# Autodesk Inventor assembly: Mark 3.5
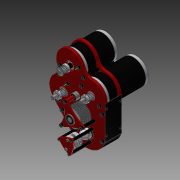
[picture p0: Inventor's stored thumbnail of the model, 180x180]
Saved by Autodesk Inventor 2013 (Build 170138000, 138)
## iProperties
Created: 2013-06-27
Part Number: Mark 3.5
Document SubType Name: Assembly
Designer: mvarma
Author: mvarma
## Documents named in this file (58)
- C:\Users\mvarma\Desktop\GRT 2013-2014 Gearbox\Mark 3\Mark 3.5.iam
- C:\Users\mvarma\Desktop\GRT 2013-2014 Gearbox\Mark 3\Plates\Mounting Plate.ipt
- C:\Users\mvarma\Desktop\GRT 2013-2014 Gearbox\Mark 3\Plates\Pnuematic Plate.ipt
- C:\Users\mvarma\Desktop\GRT 2013-2014 Gearbox\Mark 3\Plates\Main Connecting Standoff.ipt
- C:\Users\mvarma\Desktop\GRT 2013-2014 Gearbox\Mark 3\Pem Nuts\10-32 Clinch Style Pem Nut .091 Minimum Panel Thickness.ipt
- C:\Users\mvarma\Desktop\GRT 2013-2014 Gearbox\Mark 3\Bearings\FR8-2RS.ipt
- C:\Users\mvarma\Desktop\GRT 2013-2014 Gearbox\Mark 3\Bearings\FR6-2RS.ipt
- C:\Users\mvarma\Desktop\GRT 2013-2014 Gearbox\Mark 3\Encoder\Encoder Mount.ipt
- C:\Users\mvarma\Desktop\GRT 2013-2014 Gearbox\Mark 3\Encoder\S4-120-250-N-S-B.ipt
- C:\Users\mvarma\Desktop\GRT 2013-2014 Gearbox\Mark 3\Shafts\Flexible Shaft Coupler 6208K411.ipt
- C:\Users\mvarma\Desktop\GRT 2013-2014 Gearbox\Mark 3\Shafts\Cluster Shaft.ipt
- C:\Users\mvarma\Desktop\GRT 2013-2014 Gearbox\Mark 3\Spacers\Cluster Shaft Spacer.ipt
- C:\Users\mvarma\Desktop\GRT 2013-2014 Gearbox\Mark 3\Bolts\Socket Head Cap Screw 6-32 Thread 1.500 Length.ipt
- C:\Users\mvarma\Desktop\GRT 2013-2014 Gearbox\Mark 3\Gears\15T 20DP - .375 Hex Bore.ipt
- C:\Users\mvarma\Desktop\GRT 2013-2014 Gearbox\Mark 3\Gears\28T 20DP - .375 Hex Bore.ipt
- C:\Users\mvarma\Desktop\GRT 2013-2014 Gearbox\Mark 3\Bearings\FR6-2ZZ - Hex.ipt
- C:\Users\mvarma\Desktop\GRT 2013-2014 Gearbox\Mark 3\Shafts\Output Shaft.ipt
- C:\Users\mvarma\Desktop\GRT 2013-2014 Gearbox\Mark 3\Spacers\Shim 10 thou .500 Bore.ipt
- C:\Users\mvarma\Desktop\GRT 2013-2014 Gearbox\Mark 3\Bearings\R10-Open.ipt
- C:\Users\mvarma\Desktop\GRT 2013-2014 Gearbox\Mark 3\Gears\35T 20DP - .188 Ball Shifting Bore.ipt
- C:\Users\mvarma\Desktop\GRT 2013-2014 Gearbox\Mark 3\Gears\48T 20DP - .188 Ball Shifting Bore.ipt
- C:\Users\mvarma\Desktop\GRT 2013-2014 Gearbox\Mark 3\Bearings\Thrust Bearing Washer - .6250 Bore.ipt
- C:\Users\mvarma\Desktop\GRT 2013-2014 Gearbox\Mark 3\Spacers\Shim 10 thou .625 Bore.ipt
- C:\Users\mvarma\Desktop\GRT 2013-2014 Gearbox\Mark 3\Shafts\Ball Shifting Shaft.ipt
- C:\Users\mvarma\Desktop\GRT 2013-2014 Gearbox\Mark 3\Shafts\Output Shaft Insert.ipt
- C:\Users\mvarma\Desktop\GRT 2013-2014 Gearbox\Mark 3\Spacers\Shim 10 thou .375 Bore.ipt
- C:\Users\mvarma\Desktop\GRT 2013-2014 Gearbox\Mark 3\Pulleys\48T 3mm GT2 - .375 Hex Broach - Hubless.ipt
- C:\Users\mvarma\Desktop\GRT 2013-2014 Gearbox\Mark 3\Plates\Supporting Plate Standoff.ipt
- C:\Users\mvarma\Desktop\GRT 2013-2014 Gearbox\Mark 3\Bolts\Socket Head Cap Screw 10-32 Thread 3.000 Length.ipt
- C:\Users\mvarma\Desktop\GRT 2013-2014 Gearbox\Mark 3\Shafts\Tensioning Shaft.ipt
- C:\Users\mvarma\Desktop\GRT 2013-2014 Gearbox\Mark 3\Spacers\Belt Shaft Spacer 1.ipt
- C:\Users\mvarma\Desktop\GRT 2013-2014 Gearbox\Mark 3\Spacers\Belt Shaft Spacer 2.ipt
- C:\Users\mvarma\Desktop\GRT 2013-2014 Gearbox\Mark 3\Bearings\R4-2RS.ipt
- C:\Users\mvarma\Desktop\GRT 2013-2014 Gearbox\Mark 3\Bearings\R3-2RS.ipt
- C:\Users\mvarma\Desktop\GRT 2013-2014 Gearbox\Mark 3\Plates\Cim Plate.ipt
- C:\Users\mvarma\Desktop\GRT 2013-2014 Gearbox\Mark 3\Bolts\Socket Head Cap Screw 10-32 Thread 1.750 Length.ipt
- C:\Users\mvarma\Desktop\GRT 2013-2014 Gearbox\Mark 3\Motors\Mini CIM Can.ipt
- C:\Users\mvarma\Desktop\GRT 2013-2014 Gearbox\Mark 3\Motors\CIM Can.ipt
- C:\Users\mvarma\Desktop\GRT 2013-2014 Gearbox\Mark 3\Motors\Rotor.ipt
- C:\Users\mvarma\Desktop\GRT 2013-2014 Gearbox\Mark 3\Bolts\Socket Head Cap Screw 10-32 Thread .750 Length.ipt
- C:\Users\mvarma\Desktop\GRT 2013-2014 Gearbox\Mark 3\Pneumatic\FO_020_318_4F_2_03.iam
- C:\Users\mvarma\Desktop\GRT 2013-2014 Gearbox\Mark 3\Pneumatic\Mouning Standoff.ipt
- C:\Users\mvarma\Desktop\GRT 2013-2014 Gearbox\Mark 3\Pneumatic\Mounting Plate.ipt
- C:\Users\mvarma\Desktop\GRT 2013-2014 Gearbox\Mark 3\Pneumatic\Pneumatic Connector -Actuator Side.ipt
- C:\Users\mvarma\Desktop\GRT 2013-2014 Gearbox\Mark 3\Pneumatic\Pneumatic Connector -Shaft Side Cover.ipt
- C:\Users\mvarma\Desktop\GRT 2013-2014 Gearbox\Mark 3\Pem Nuts\4-40 Clinch Style Pem Nut .091 Minimum Panel Thickness.ipt
- C:\Users\mvarma\Desktop\GRT 2013-2014 Gearbox\Mark 3\Bolts\Socket Head Cap Screw 4-40 Thread 1.000 Length.ipt
- C:\Users\mvarma\Desktop\GRT 2013-2014 Gearbox\Mark 3\.0625 Spring Pin .2500 Long.ipt
- C:\Users\mvarma\Desktop\GRT 2013-2014 Gearbox\Mark 3\Bolts\Button Head Cap Screw 4-40 Thread .125 Length.ipt
- C:\Users\mvarma\Desktop\GRT 2013-2014 Gearbox\Mark 3\Bolts\Socket Head Cap Screw 8-32 Thread .375 Length.ipt
- C:\Users\mvarma\Desktop\GRT 2013-2014 Gearbox\Mark 3\Bolts\Socket Head Cap Screw 6-32 Thread 2.250 Length.ipt
- C:\Users\mvarma\Desktop\GRT 2013-2014 Gearbox\Mark 3\Pulleys\16T 3mm GT2 - 8mm Key Broach.ipt
- C:\Users\mvarma\Desktop\GRT 2013-2014 Gearbox\Mark 3\Spacers\Cim Spacer.ipt
- C:\Users\mvarma\Desktop\GRT 2013-2014 Gearbox\Mark 3\Spacers\MiniCim Spacer.ipt
- C:\Users\mvarma\Desktop\GRT 2013-2014 Gearbox\Mark 3\Pem Nuts\.25-20 Clinch Style Pem Nut .125 Minimum Panel Thickness.ipt
- C:\Users\mvarma\Desktop\GRT 2013-2014 Gearbox\Mark 3\Frame Segment.ipt
- C:\Users\mvarma\Desktop\GRT 2013-2014 Gearbox\Mark 3\Plates\Sheild.ipt
- C:\Users\mvarma\Desktop\GRT 2013-2014 Gearbox\Mark 3\Plates\Sheild - Upper.ipt
## Components (116 placed, 56 different names)
1. 10-32 Clinch Style Pem Nut .091 Minimum Panel Thickness:1 — Mate:24, Mate:31
2. 10-32 Clinch Style Pem Nut .091 Minimum Panel Thickness:2 — Mate:27, Mate:28
3. 10-32 Clinch Style Pem Nut .091 Minimum Panel Thickness:3 — Mate:26, Mate:30
4. 10-32 Clinch Style Pem Nut .091 Minimum Panel Thickness:4 — Mate:33, Mate:238
5. 10-32 Clinch Style Pem Nut .091 Minimum Panel Thickness:5 — Mate:20, Mate:36
6. 10-32 Clinch Style Pem Nut .091 Minimum Panel Thickness:6 — Mate:21, Mate:34
7. 10-32 Clinch Style Pem Nut .091 Minimum Panel Thickness:7 — Mate:23, Mate:29
8. 10-32 Clinch Style Pem Nut .091 Minimum Panel Thickness:8 — Mate:35, Mate:239
9. 10-32 Clinch Style Pem Nut .091 Minimum Panel Thickness:9 — Mate:25, Mate:32
10. FR8-2RS:1 — Mate:37, Mate:40, Mate:65, Mate:67
11. FR6-2RS:1 — Mate:38, Mate:39, Mate:51
12. Encoder Mount:1 — Mate:41, Mate:42, Mate:43, Mate:44, Mate:45, Mate:52, Mate:53, Mate:54, Mate:55
13. S4-120-250-N-S-B:1 — Mate:44, Mate:45, Mate:46, Mate:47, Mate:48
14. Flexible Shaft Coupler 6208K411:1 — Mate:46, Mate:47, Mate:49
15. Cluster Shaft:1 — Mate:48, Mate:49, Mate:50, Mate:56, Mate:57, Mate:58, Mate:59, Mate:62, Mate:63, Mate:88, Mate:90, Mate:91, Mate:92, Mate:93, Mate:94, Mate:95, Mate:98
16. Cluster Shaft Spacer:1 — Mate:50, Mate:51, Mate:60
17. Socket Head Cap Screw 6-32 Thread 1.500 Length:1 — Mate:52, Mate:55
18. Socket Head Cap Screw 6-32 Thread 1.500 Length:2 — Mate:53, Mate:54
19. 15T 20DP - .375 Hex Bore:1 — Mate:56, Mate:58, Mate:61, Mate:64
20. 28T 20DP - .375 Hex Bore:1 — Mate:57, Mate:59, Mate:60, Mate:61
21. FR6-2ZZ - Hex:1 — Mate:62, Mate:63, Mate:64, Mate:89
22. Output Shaft:1 — Mate:65, Mate:66, Mate:68, Mate:69, Mate:71, Mate:72, Mate:74, Mate:76, Mate:79, Mate:81, Mate:83, Mate:84, Mate:86, Mate:87, Mate:235
23. Shim 10 thou .500 Bore:1 — Mate:66, Mate:67, Mate:68, Mate:70
24. R10-Open:1 — Mate:69, Mate:70, Mate:73
25. R10-Open:2 — Mate:76, Mate:77, Mate:78
26. 35T 20DP - .188 Ball Shifting Bore:1 — Mate:71, Mate:73, Mate:75
27. 48T 20DP - .188 Ball Shifting Bore:1 — Mate:72, Mate:78, Mate:80
28. Thrust Bearing Washer - .6250 Bore:1 — Mate:79, Mate:80, Mate:82
29. Thrust Bearing Washer - .6250 Bore:2 — Mate:74, Mate:75, Mate:77
30. Shim 10 thou .625 Bore:1 — Mate:81, Mate:82
31. Ball Shifting Shaft:1 — Mate:85, Flush:1, Mate:123, Mate:124, Mate:196, Mate:198, Mate:199
32. Output Shaft Insert:1 — Mate:83, Mate:84, Mate:85, Flush:1
33. FR8-2RS:2 — Mate:86, Mate:87
34. Shim 10 thou .500 Bore:2 — Mate:88, Mate:89, Mate:96
35. Shim 10 thou .375 Bore:1 — Mate:90, Mate:91, Mate:99
36. 48T 3mm GT2 - .375 Hex Broach - Hubless:1 — Mate:93, Mate:95, Mate:97, Flush:2
37. 48T 3mm GT2 - .375 Hex Broach - Hubless:2 — Mate:92, Mate:94, Mate:96, Mate:97, Mate:223, Mate:224
38. FR6-2RS:2 — Mate:98, Mate:99, Mate:100, Mate:101
39. Supporting Plate Standoff:1 — Mate:103, Mate:106
40. Supporting Plate Standoff:2 — Mate:104, Mate:105
41. Socket Head Cap Screw 10-32 Thread 3.000 Length:1 — Mate:108, Mate:109
42. Socket Head Cap Screw 10-32 Thread 3.000 Length:2 — Mate:111, Mate:112, Mate:113
43. Socket Head Cap Screw 10-32 Thread 3.000 Length:3 — Mate:107, Mate:110
44. Tensioning Shaft:1 — Mate:113, Mate:114, Mate:115, Mate:116, Mate:117, Mate:118
45. Belt Shaft Spacer 1:1 — Mate:115, Mate:120
46. Belt Shaft Spacer 2:1 — Mate:116, Mate:121, Mate:122
47. R4-2RS:1 — Mate:118, Mate:119, Mate:120
48. R4-2RS:2 — Mate:117, Mate:119, Mate:121
49. R3-2RS:1 — Mate:123, Mate:124, Mate:200
50. Cim Plate:1 — Mate:127, Mate:128, Mate:129, Mate:130, Mate:131, Mate:132, Mate:133, Mate:134, Mate:135, Mate:136, Mate:137, Mate:138, Mate:139, Mate:140, Mate:141, Mate:142, Mate:143, Mate:144, Mate:145, Mate:146, Mate:147, Mate:148, Mate:149, Mate:150, Mate:151, Mate:152, Mate:153, Mate:154, Mate:155, Mate:162, Mate:163, Mate:164, Mate:165, Mate:166, Mate:167, Mate:168, Mate:169, Mate:170, Mate:171, Mate:172, Mate:173, Mate:174, Mate:175, Mate:176, Mate:177, Mate:178, Mate:179, Mate:242, Mate:243, Flush:3, Mate:244, Mate:246, Mate:250, Mate:254, Mate:258
51. Socket Head Cap Screw 10-32 Thread 1.750 Length:1 — Mate:135, Mate:143
52. Socket Head Cap Screw 10-32 Thread 1.750 Length:2 — Mate:137, Mate:142
53. Socket Head Cap Screw 10-32 Thread 1.750 Length:3 — Mate:136, Mate:144
54. Socket Head Cap Screw 10-32 Thread 1.750 Length:4 — Mate:138, Mate:141
55. Socket Head Cap Screw 10-32 Thread 1.750 Length:5 — Mate:139, Mate:146
56. Socket Head Cap Screw 10-32 Thread 1.750 Length:6 — Mate:140, Mate:145
57. Mini CIM Can:1 — Mate:147, Mate:148, Mate:149, Mate:156, Mate:161, Mate:230
58. CIM Can:1 — Mate:150, Mate:151, Mate:152, Mate:157, Mate:159, Mate:228
59. CIM Can:2 — Mate:153, Mate:154, Mate:155, Mate:158, Mate:160, Mate:229
60. Rotor:1 — Mate:158, Mate:160, Mate:220, Mate:225
61. Rotor:2 — Mate:157, Mate:159, Mate:222, Mate:226
62. Rotor:3 — Mate:156, Mate:161, Mate:221, Mate:227
63. Socket Head Cap Screw 10-32 Thread .750 Length:1 — Mate:162, Mate:169
64. Socket Head Cap Screw 10-32 Thread .750 Length:2 — Mate:163, Mate:168
65. Socket Head Cap Screw 10-32 Thread .750 Length:3 — Mate:165, Mate:172
66. Socket Head Cap Screw 10-32 Thread .750 Length:4 — Mate:166, Mate:170
67. Socket Head Cap Screw 10-32 Thread .750 Length:5 — Mate:167, Mate:173
68. Socket Head Cap Screw 10-32 Thread .750 Length:6 — Mate:164, Mate:171
69. FO_020_318_4F_2_03:1 [sub-assembly] — Mate:184, Mate:185, Mate:190, Mate:191, Mate:192, Mate:193, Mate:205, Mate:212, Mate:213
70. Mouning Standoff:1 — Mate:176, Mate:177, Mate:182, Mate:183
71. Mounting Plate:2 — Mate:180, Mate:181, Mate:182, Mate:183, Mate:184, Mate:185, Mate:186, Mate:187, Mate:188, Mate:189, Mate:213, Mate:214, Mate:215, Mate:216, Mate:217, Mate:218, Mate:219
72. Pneumatic Connector -Actuator Side:1 — Mate:194, Mate:195, Mate:197, Mate:200, Mate:205, Mate:206, Mate:207, Mate:208, Mate:210, Mate:212
73. Pneumatic Connector -Shaft Side Cover:1 — Mate:194, Mate:195, Mate:196, Mate:197, Mate:209, Mate:211
74. Mouning Standoff:2 — Mate:175, Mate:178, Mate:181
75. Mouning Standoff:3 — Mate:174, Mate:179, Mate:180
76. 4-40 Clinch Style Pem Nut .091 Minimum Panel Thickness:1 — Mate:187, Mate:188
77. 4-40 Clinch Style Pem Nut .091 Minimum Panel Thickness:2 — Mate:186, Mate:189
78. Socket Head Cap Screw 4-40 Thread 1.000 Length:1 — Mate:191, Mate:192
79. Socket Head Cap Screw 4-40 Thread 1.000 Length:2 — Mate:190, Mate:193
80. .0625 Spring Pin .2500 Long:1 — Mate:198, Mate:199
81. Socket Head Cap Screw 8-32 Thread .375 Length:1 — Mate:206, Mate:207
82. Button Head Cap Screw 4-40 Thread .125 Length:1 — Mate:208, Mate:209
83. Button Head Cap Screw 4-40 Thread .125 Length:2 — Mate:210, Mate:211
84. Socket Head Cap Screw 6-32 Thread 2.250 Length:1 — Mate:216, Mate:219
85. Socket Head Cap Screw 6-32 Thread 2.250 Length:2 — Mate:215, Mate:217
86. Socket Head Cap Screw 6-32 Thread 2.250 Length:3 — Mate:214, Mate:218
87. 16T 3mm GT2 - 8mm Key Broach:1 — Mate:221, Flush:2
88. 16T 3mm GT2 - 8mm Key Broach:2 — Mate:222, Mate:224
89. 16T 3mm GT2 - 8mm Key Broach:3 — Mate:220, Mate:223
90. Cim Spacer:1 — Mate:225, Mate:229
91. MiniCim Spacer:1 — Mate:227, Mate:230
92. Cim Spacer:2 — Mate:226, Mate:228
93. .25-20 Clinch Style Pem Nut .125 Minimum Panel Thickness:1 — Mate:231, Mate:233
94. .25-20 Clinch Style Pem Nut .125 Minimum Panel Thickness:2 — Mate:232, Mate:234
95. Frame Segment:1 — Mate:235, Mate:236, Mate:237
96. Sheild:1 — Mate:242, Mate:243, Flush:3, Mate:244, Mate:247, Mate:248, Mate:251, Mate:252, Mate:255, Mate:256, Mate:259, Mate:260, Mate:261, Flush:4, Mate:262
97. Button Head Cap Screw 4-40 Thread .125 Length:3 — Mate:249, Mate:252
98. Button Head Cap Screw 4-40 Thread .125 Length:4 — Mate:246, Mate:247
99. Button Head Cap Screw 4-40 Thread .125 Length:5 — Mate:257, Mate:259
100. Button Head Cap Screw 4-40 Thread .125 Length:6 — Mate:250, Mate:251
101. Button Head Cap Screw 4-40 Thread .125 Length:7 — Mate:245, Mate:248
102. Button Head Cap Screw 4-40 Thread .125 Length:8 — Mate:253, Mate:255
103. Button Head Cap Screw 4-40 Thread .125 Length:9 — Mate:258, Mate:260
104. Button Head Cap Screw 4-40 Thread .125 Length:10 — Mate:254, Mate:256
105. Sheild - Upper:1 — Mate:261, Flush:4, Mate:262
106. Mounting Plate:1 — Mate:1, Mate:2, Mate:3, Mate:5, Mate:7, Mate:8, Mate:9, Mate:10, Mate:11, Mate:12, Mate:13, Mate:14, Mate:15, Mate:16, Mate:17, Mate:18, Mate:20, Mate:21, Mate:23, Mate:24, Mate:25, Mate:26, Mate:27, Mate:28, Mate:29, Mate:30, Mate:31, Mate:32, Mate:33, Mate:34, Mate:35, Mate:36, Mate:37, Mate:38, Mate:39, Mate:40, Mate:41, Mate:42, Mate:43, Mate:231, Mate:232, Mate:233, Mate:234, Mate:236, Mate:237, Mate:238, Mate:239, Mate:240, Mate:241, Mate:245, Mate:249, Mate:253, Mate:257
107. Pnuematic Plate:1 — Mate:100, Mate:101, Mate:102, Mate:103, Mate:104, Mate:105, Mate:106, Mate:107, Mate:108, Mate:109, Mate:110, Mate:111, Mate:112, Mate:114, Mate:122
108. Main Connecting Standoff:1 — Mate:3, Mate:16, Mate:102
109. Main Connecting Standoff:2 — Mate:2, Mate:17
110. Main Connecting Standoff:3 — Mate:1, Mate:18, Mate:129
111. Main Connecting Standoff:4 — Mate:8, Mate:12, Mate:132
112. Main Connecting Standoff:5 — Mate:7, Mate:11
113. Main Connecting Standoff:6 — Mate:9, Mate:10, Mate:127, Mate:133, Mate:134
114. Main Connecting Standoff:7 — Mate:5, Mate:14
115. Main Connecting Standoff:8 — Mate:15, Mate:128, Mate:130, Mate:240
116. Main Connecting Standoff:9 — Mate:13, Mate:131, Mate:241
## Relationships (256: Mate 252, Flush 4)
- Mate:1: Mounting Plate:1 ↔ Main Connecting Standoff:3
- Mate:2: Mounting Plate:1 ↔ Main Connecting Standoff:2
- Mate:3: Mounting Plate:1 ↔ Main Connecting Standoff:1
- Mate:5: Mounting Plate:1 ↔ Main Connecting Standoff:7
- Mate:7: Mounting Plate:1 ↔ Main Connecting Standoff:5
- Mate:8: Mounting Plate:1 ↔ Main Connecting Standoff:4
- Mate:9: Mounting Plate:1 ↔ Main Connecting Standoff:6
- Mate:10: Mounting Plate:1 ↔ Main Connecting Standoff:6
- Mate:11: Mounting Plate:1 ↔ Main Connecting Standoff:5
- Mate:12: Mounting Plate:1 ↔ Main Connecting Standoff:4
- Mate:13: Mounting Plate:1 ↔ Main Connecting Standoff:9
- Mate:14: Mounting Plate:1 ↔ Main Connecting Standoff:7
- Mate:15: Mounting Plate:1 ↔ Main Connecting Standoff:8
- Mate:16: Mounting Plate:1 ↔ Main Connecting Standoff:1
- Mate:17: Mounting Plate:1 ↔ Main Connecting Standoff:2
- Mate:18: Mounting Plate:1 ↔ Main Connecting Standoff:3
- Mate:20: 10-32 Clinch Style Pem Nut .091 Minimum Panel Thickness:5 ↔ Mounting Plate:1
- Mate:21: 10-32 Clinch Style Pem Nut .091 Minimum Panel Thickness:6 ↔ Mounting Plate:1
- Mate:23: 10-32 Clinch Style Pem Nut .091 Minimum Panel Thickness:7 ↔ Mounting Plate:1
- Mate:24: 10-32 Clinch Style Pem Nut .091 Minimum Panel Thickness:1 ↔ Mounting Plate:1
- Mate:25: 10-32 Clinch Style Pem Nut .091 Minimum Panel Thickness:9 ↔ Mounting Plate:1
- Mate:26: 10-32 Clinch Style Pem Nut .091 Minimum Panel Thickness:3 ↔ Mounting Plate:1
- Mate:27: 10-32 Clinch Style Pem Nut .091 Minimum Panel Thickness:2 ↔ Mounting Plate:1
- Mate:28: 10-32 Clinch Style Pem Nut .091 Minimum Panel Thickness:2 ↔ Mounting Plate:1
- Mate:29: 10-32 Clinch Style Pem Nut .091 Minimum Panel Thickness:7 ↔ Mounting Plate:1
- Mate:30: 10-32 Clinch Style Pem Nut .091 Minimum Panel Thickness:3 ↔ Mounting Plate:1
- Mate:31: 10-32 Clinch Style Pem Nut .091 Minimum Panel Thickness:1 ↔ Mounting Plate:1
- Mate:32: 10-32 Clinch Style Pem Nut .091 Minimum Panel Thickness:9 ↔ Mounting Plate:1
- Mate:33: 10-32 Clinch Style Pem Nut .091 Minimum Panel Thickness:4 ↔ Mounting Plate:1
- Mate:34: 10-32 Clinch Style Pem Nut .091 Minimum Panel Thickness:6 ↔ Mounting Plate:1
- Mate:35: 10-32 Clinch Style Pem Nut .091 Minimum Panel Thickness:8 ↔ Mounting Plate:1
- Mate:36: 10-32 Clinch Style Pem Nut .091 Minimum Panel Thickness:5 ↔ Mounting Plate:1
- Mate:37: FR8-2RS:1 ↔ Mounting Plate:1
- Mate:38: FR6-2RS:1 ↔ Mounting Plate:1
- Mate:39: FR6-2RS:1 ↔ Mounting Plate:1
- Mate:40: FR8-2RS:1 ↔ Mounting Plate:1
- Mate:41: Encoder Mount:1 ↔ Mounting Plate:1
- Mate:42: Encoder Mount:1 ↔ Mounting Plate:1
- Mate:43: Encoder Mount:1 ↔ Mounting Plate:1
- Mate:44: Encoder Mount:1 ↔ S4-120-250-N-S-B:1
- Mate:45: Encoder Mount:1 ↔ S4-120-250-N-S-B:1
- Mate:46: S4-120-250-N-S-B:1 ↔ Flexible Shaft Coupler 6208K411:1
- Mate:47: S4-120-250-N-S-B:1 ↔ Flexible Shaft Coupler 6208K411:1
- Mate:48: S4-120-250-N-S-B:1 ↔ Cluster Shaft:1
- Mate:49: Flexible Shaft Coupler 6208K411:1 ↔ Cluster Shaft:1
- Mate:50: Cluster Shaft:1 ↔ Cluster Shaft Spacer:1
- Mate:51: FR6-2RS:1 ↔ Cluster Shaft Spacer:1
- Mate:52: Encoder Mount:1 ↔ Socket Head Cap Screw 6-32 Thread 1.500 Length:1
- Mate:53: Encoder Mount:1 ↔ Socket Head Cap Screw 6-32 Thread 1.500 Length:2
- Mate:54: Encoder Mount:1 ↔ Socket Head Cap Screw 6-32 Thread 1.500 Length:2
- Mate:55: Encoder Mount:1 ↔ Socket Head Cap Screw 6-32 Thread 1.500 Length:1
- Mate:56: Cluster Shaft:1 ↔ 15T 20DP - .375 Hex Bore:1
- Mate:57: Cluster Shaft:1 ↔ 28T 20DP - .375 Hex Bore:1
- Mate:58: Cluster Shaft:1 ↔ 15T 20DP - .375 Hex Bore:1
- Mate:59: Cluster Shaft:1 ↔ 28T 20DP - .375 Hex Bore:1
- Mate:60: Cluster Shaft Spacer:1 ↔ 28T 20DP - .375 Hex Bore:1
- Mate:61: 15T 20DP - .375 Hex Bore:1 ↔ 28T 20DP - .375 Hex Bore:1
- Mate:62: Cluster Shaft:1 ↔ FR6-2ZZ - Hex:1
- Mate:63: Cluster Shaft:1 ↔ FR6-2ZZ - Hex:1
- Mate:64: 15T 20DP - .375 Hex Bore:1 ↔ FR6-2ZZ - Hex:1
- Mate:65: FR8-2RS:1 ↔ Output Shaft:1
- Mate:66: Output Shaft:1 ↔ Shim 10 thou .500 Bore:1
- Mate:67: FR8-2RS:1 ↔ Shim 10 thou .500 Bore:1
- Mate:68: Output Shaft:1 ↔ Shim 10 thou .500 Bore:1
- Mate:69: Output Shaft:1 ↔ R10-Open:1
- Mate:70: Shim 10 thou .500 Bore:1 ↔ R10-Open:1
- Mate:71: Output Shaft:1 ↔ 35T 20DP - .188 Ball Shifting Bore:1
- Mate:72: Output Shaft:1 ↔ 48T 20DP - .188 Ball Shifting Bore:1
- Mate:73: R10-Open:1 ↔ 35T 20DP - .188 Ball Shifting Bore:1
- Mate:74: Output Shaft:1 ↔ Thrust Bearing Washer - .6250 Bore:2
- Mate:75: 35T 20DP - .188 Ball Shifting Bore:1 ↔ Thrust Bearing Washer - .6250 Bore:2
- Mate:76: Output Shaft:1 ↔ R10-Open:2
- Mate:77: R10-Open:2 ↔ Thrust Bearing Washer - .6250 Bore:2
- Mate:78: R10-Open:2 ↔ 48T 20DP - .188 Ball Shifting Bore:1
- Mate:79: Output Shaft:1 ↔ Thrust Bearing Washer - .6250 Bore:1
- Mate:80: 48T 20DP - .188 Ball Shifting Bore:1 ↔ Thrust Bearing Washer - .6250 Bore:1
- Mate:81: Output Shaft:1 ↔ Shim 10 thou .625 Bore:1
- Mate:82: Thrust Bearing Washer - .6250 Bore:1 ↔ Shim 10 thou .625 Bore:1
- Mate:83: Output Shaft:1 ↔ Output Shaft Insert:1
- Mate:84: Output Shaft:1 ↔ Output Shaft Insert:1
- Mate:85: Ball Shifting Shaft:1 ↔ Output Shaft Insert:1
- Flush:1: Ball Shifting Shaft:1 ↔ Output Shaft Insert:1
- Mate:86: Output Shaft:1 ↔ FR8-2RS:2
- Mate:87: Output Shaft:1 ↔ FR8-2RS:2
- Mate:88: Cluster Shaft:1 ↔ Shim 10 thou .500 Bore:2
- Mate:89: FR6-2ZZ - Hex:1 ↔ Shim 10 thou .500 Bore:2
- Mate:90: Cluster Shaft:1 ↔ Shim 10 thou .375 Bore:1
- Mate:91: Cluster Shaft:1 ↔ Shim 10 thou .375 Bore:1
- Mate:92: Cluster Shaft:1 ↔ 48T 3mm GT2 - .375 Hex Broach - Hubless:2
- Mate:93: Cluster Shaft:1 ↔ 48T 3mm GT2 - .375 Hex Broach - Hubless:1
- Mate:94: Cluster Shaft:1 ↔ 48T 3mm GT2 - .375 Hex Broach - Hubless:2
- Mate:95: Cluster Shaft:1 ↔ 48T 3mm GT2 - .375 Hex Broach - Hubless:1
- Mate:96: Shim 10 thou .500 Bore:2 ↔ 48T 3mm GT2 - .375 Hex Broach - Hubless:2
- Mate:97: 48T 3mm GT2 - .375 Hex Broach - Hubless:1 ↔ 48T 3mm GT2 - .375 Hex Broach - Hubless:2
- Mate:98: Cluster Shaft:1 ↔ FR6-2RS:2
- Mate:99: Shim 10 thou .375 Bore:1 ↔ FR6-2RS:2
- Mate:100: FR6-2RS:2 ↔ Pnuematic Plate:1
- Mate:101: FR6-2RS:2 ↔ Pnuematic Plate:1
- Mate:102: Pnuematic Plate:1 ↔ Main Connecting Standoff:1
- Mate:103: Supporting Plate Standoff:1 ↔ Pnuematic Plate:1
- Mate:104: Supporting Plate Standoff:2 ↔ Pnuematic Plate:1
- Mate:105: Supporting Plate Standoff:2 ↔ Pnuematic Plate:1
- Mate:106: Supporting Plate Standoff:1 ↔ Pnuematic Plate:1
- Mate:107: Socket Head Cap Screw 10-32 Thread 3.000 Length:3 ↔ Pnuematic Plate:1
- Mate:108: Socket Head Cap Screw 10-32 Thread 3.000 Length:1 ↔ Pnuematic Plate:1
- Mate:109: Socket Head Cap Screw 10-32 Thread 3.000 Length:1 ↔ Pnuematic Plate:1
- Mate:110: Socket Head Cap Screw 10-32 Thread 3.000 Length:3 ↔ Pnuematic Plate:1
- Mate:111: Socket Head Cap Screw 10-32 Thread 3.000 Length:2 ↔ Pnuematic Plate:1
- Mate:112: Socket Head Cap Screw 10-32 Thread 3.000 Length:2 ↔ Pnuematic Plate:1
- Mate:113: Socket Head Cap Screw 10-32 Thread 3.000 Length:2 ↔ Tensioning Shaft:1
- Mate:114: Tensioning Shaft:1 ↔ Pnuematic Plate:1
- Mate:115: Tensioning Shaft:1 ↔ Belt Shaft Spacer 1:1
- Mate:116: Tensioning Shaft:1 ↔ Belt Shaft Spacer 2:1
- Mate:117: Tensioning Shaft:1 ↔ R4-2RS:2
- Mate:118: Tensioning Shaft:1 ↔ R4-2RS:1
- Mate:119: R4-2RS:1 ↔ R4-2RS:2
- Mate:120: Belt Shaft Spacer 1:1 ↔ R4-2RS:1
- Mate:121: Belt Shaft Spacer 2:1 ↔ R4-2RS:2
- Mate:122: Belt Shaft Spacer 2:1 ↔ Pnuematic Plate:1
- Mate:123: Ball Shifting Shaft:1 ↔ R3-2RS:1
- Mate:124: Ball Shifting Shaft:1 ↔ R3-2RS:1
- Mate:127: Cim Plate:1 ↔ Main Connecting Standoff:6
- Mate:128: Cim Plate:1 ↔ Main Connecting Standoff:8
- Mate:129: Cim Plate:1 ↔ Main Connecting Standoff:3
- Mate:130: Cim Plate:1 ↔ Main Connecting Standoff:8
- Mate:131: Cim Plate:1 ↔ Main Connecting Standoff:9
- Mate:132: Cim Plate:1 ↔ Main Connecting Standoff:4
- Mate:133: Cim Plate:1 ↔ Main Connecting Standoff:6
- Mate:134: Cim Plate:1 ↔ Main Connecting Standoff:6
- Mate:135: Cim Plate:1 ↔ Socket Head Cap Screw 10-32 Thread 1.750 Length:1
- Mate:136: Cim Plate:1 ↔ Socket Head Cap Screw 10-32 Thread 1.750 Length:3
- Mate:137: Cim Plate:1 ↔ Socket Head Cap Screw 10-32 Thread 1.750 Length:2
- Mate:138: Cim Plate:1 ↔ Socket Head Cap Screw 10-32 Thread 1.750 Length:4
- Mate:139: Cim Plate:1 ↔ Socket Head Cap Screw 10-32 Thread 1.750 Length:5
- Mate:140: Cim Plate:1 ↔ Socket Head Cap Screw 10-32 Thread 1.750 Length:6
- Mate:141: Cim Plate:1 ↔ Socket Head Cap Screw 10-32 Thread 1.750 Length:4
- Mate:142: Cim Plate:1 ↔ Socket Head Cap Screw 10-32 Thread 1.750 Length:2
- Mate:143: Cim Plate:1 ↔ Socket Head Cap Screw 10-32 Thread 1.750 Length:1
- Mate:144: Cim Plate:1 ↔ Socket Head Cap Screw 10-32 Thread 1.750 Length:3
- Mate:145: Cim Plate:1 ↔ Socket Head Cap Screw 10-32 Thread 1.750 Length:6
- Mate:146: Cim Plate:1 ↔ Socket Head Cap Screw 10-32 Thread 1.750 Length:5
- Mate:147: Cim Plate:1 ↔ Mini CIM Can:1
- Mate:148: Cim Plate:1 ↔ Mini CIM Can:1
- Mate:149: Cim Plate:1 ↔ Mini CIM Can:1
- Mate:150: Cim Plate:1 ↔ CIM Can:1
- Mate:151: Cim Plate:1 ↔ CIM Can:1
- Mate:152: Cim Plate:1 ↔ CIM Can:1
- Mate:153: Cim Plate:1 ↔ CIM Can:2
- Mate:154: Cim Plate:1 ↔ CIM Can:2
- Mate:155: Cim Plate:1 ↔ CIM Can:2
- Mate:156: Mini CIM Can:1 ↔ Rotor:3
- Mate:157: CIM Can:1 ↔ Rotor:2
- Mate:158: CIM Can:2 ↔ Rotor:1
- Mate:159: CIM Can:1 ↔ Rotor:2
- Mate:160: CIM Can:2 ↔ Rotor:1
- Mate:161: Mini CIM Can:1 ↔ Rotor:3
- Mate:162: Cim Plate:1 ↔ Socket Head Cap Screw 10-32 Thread .750 Length:1
- Mate:163: Cim Plate:1 ↔ Socket Head Cap Screw 10-32 Thread .750 Length:2
- Mate:164: Cim Plate:1 ↔ Socket Head Cap Screw 10-32 Thread .750 Length:6
- Mate:165: Cim Plate:1 ↔ Socket Head Cap Screw 10-32 Thread .750 Length:3
- Mate:166: Cim Plate:1 ↔ Socket Head Cap Screw 10-32 Thread .750 Length:4
- Mate:167: Cim Plate:1 ↔ Socket Head Cap Screw 10-32 Thread .750 Length:5
- Mate:168: Cim Plate:1 ↔ Socket Head Cap Screw 10-32 Thread .750 Length:2
- Mate:169: Cim Plate:1 ↔ Socket Head Cap Screw 10-32 Thread .750 Length:1
- Mate:170: Cim Plate:1 ↔ Socket Head Cap Screw 10-32 Thread .750 Length:4
- Mate:171: Cim Plate:1 ↔ Socket Head Cap Screw 10-32 Thread .750 Length:6
- Mate:172: Cim Plate:1 ↔ Socket Head Cap Screw 10-32 Thread .750 Length:3
- Mate:173: Cim Plate:1 ↔ Socket Head Cap Screw 10-32 Thread .750 Length:5
- Mate:174: Cim Plate:1 ↔ Mouning Standoff:3
- Mate:175: Cim Plate:1 ↔ Mouning Standoff:2
- Mate:176: Cim Plate:1 ↔ Mouning Standoff:1
- Mate:177: Cim Plate:1 ↔ Mouning Standoff:1
- Mate:178: Cim Plate:1 ↔ Mouning Standoff:2
- Mate:179: Cim Plate:1 ↔ Mouning Standoff:3
- Mate:180: Mounting Plate:2 ↔ Mouning Standoff:3
- Mate:181: Mounting Plate:2 ↔ Mouning Standoff:2
- Mate:182: Mouning Standoff:1 ↔ Mounting Plate:2
- Mate:183: Mouning Standoff:1 ↔ Mounting Plate:2
- Mate:184: FO_020_318_4F_2_03:1 ↔ Mounting Plate:2
- Mate:185: FO_020_318_4F_2_03:1 ↔ Mounting Plate:2
- Mate:186: Mounting Plate:2 ↔ 4-40 Clinch Style Pem Nut .091 Minimum Panel Thickness:2
- Mate:187: Mounting Plate:2 ↔ 4-40 Clinch Style Pem Nut .091 Minimum Panel Thickness:1
- Mate:188: Mounting Plate:2 ↔ 4-40 Clinch Style Pem Nut .091 Minimum Panel Thickness:1
- Mate:189: Mounting Plate:2 ↔ 4-40 Clinch Style Pem Nut .091 Minimum Panel Thickness:2
- Mate:190: FO_020_318_4F_2_03:1 ↔ Socket Head Cap Screw 4-40 Thread 1.000 Length:2
- Mate:191: FO_020_318_4F_2_03:1 ↔ Socket Head Cap Screw 4-40 Thread 1.000 Length:1
- Mate:192: FO_020_318_4F_2_03:1 ↔ Socket Head Cap Screw 4-40 Thread 1.000 Length:1
- Mate:193: FO_020_318_4F_2_03:1 ↔ Socket Head Cap Screw 4-40 Thread 1.000 Length:2
- Mate:194: Pneumatic Connector -Actuator Side:1 ↔ Pneumatic Connector -Shaft Side Cover:1
- Mate:195: Pneumatic Connector -Actuator Side:1 ↔ Pneumatic Connector -Shaft Side Cover:1
- Mate:196: Ball Shifting Shaft:1 ↔ Pneumatic Connector -Shaft Side Cover:1
- Mate:197: Pneumatic Connector -Actuator Side:1 ↔ Pneumatic Connector -Shaft Side Cover:1
- Mate:198: Ball Shifting Shaft:1 ↔ .0625 Spring Pin .2500 Long:1
- Mate:199: Ball Shifting Shaft:1 ↔ .0625 Spring Pin .2500 Long:1
- Mate:200: R3-2RS:1 ↔ Pneumatic Connector -Actuator Side:1
- Mate:205: FO_020_318_4F_2_03:1 ↔ Pneumatic Connector -Actuator Side:1
- Mate:206: Pneumatic Connector -Actuator Side:1 ↔ Socket Head Cap Screw 8-32 Thread .375 Length:1
- Mate:207: Pneumatic Connector -Actuator Side:1 ↔ Socket Head Cap Screw 8-32 Thread .375 Length:1
- Mate:208: Pneumatic Connector -Actuator Side:1 ↔ Button Head Cap Screw 4-40 Thread .125 Length:1
- Mate:209: Pneumatic Connector -Shaft Side Cover:1 ↔ Button Head Cap Screw 4-40 Thread .125 Length:1
- Mate:210: Pneumatic Connector -Actuator Side:1 ↔ Button Head Cap Screw 4-40 Thread .125 Length:2
- Mate:211: Pneumatic Connector -Shaft Side Cover:1 ↔ Button Head Cap Screw 4-40 Thread .125 Length:2
- Mate:212: FO_020_318_4F_2_03:1 ↔ Pneumatic Connector -Actuator Side:1
- Mate:213: FO_020_318_4F_2_03:1 ↔ Mounting Plate:2
- Mate:214: Mounting Plate:2 ↔ Socket Head Cap Screw 6-32 Thread 2.250 Length:3
- Mate:215: Mounting Plate:2 ↔ Socket Head Cap Screw 6-32 Thread 2.250 Length:2
- Mate:216: Mounting Plate:2 ↔ Socket Head Cap Screw 6-32 Thread 2.250 Length:1
- Mate:217: Mounting Plate:2 ↔ Socket Head Cap Screw 6-32 Thread 2.250 Length:2
- Mate:218: Mounting Plate:2 ↔ Socket Head Cap Screw 6-32 Thread 2.250 Length:3
- Mate:219: Mounting Plate:2 ↔ Socket Head Cap Screw 6-32 Thread 2.250 Length:1
- Mate:220: Rotor:1 ↔ 16T 3mm GT2 - 8mm Key Broach:3
- Mate:221: Rotor:3 ↔ 16T 3mm GT2 - 8mm Key Broach:1
- Mate:222: Rotor:2 ↔ 16T 3mm GT2 - 8mm Key Broach:2
- Mate:223: 48T 3mm GT2 - .375 Hex Broach - Hubless:2 ↔ 16T 3mm GT2 - 8mm Key Broach:3
- Mate:224: 48T 3mm GT2 - .375 Hex Broach - Hubless:2 ↔ 16T 3mm GT2 - 8mm Key Broach:2
- Flush:2: 48T 3mm GT2 - .375 Hex Broach - Hubless:1 ↔ 16T 3mm GT2 - 8mm Key Broach:1
- Mate:225: Rotor:1 ↔ Cim Spacer:1
- Mate:226: Rotor:2 ↔ Cim Spacer:2
- Mate:227: Rotor:3 ↔ MiniCim Spacer:1
- Mate:228: CIM Can:1 ↔ Cim Spacer:2
- Mate:229: CIM Can:2 ↔ Cim Spacer:1
- Mate:230: Mini CIM Can:1 ↔ MiniCim Spacer:1
- Mate:231: .25-20 Clinch Style Pem Nut .125 Minimum Panel Thickness:1 ↔ Mounting Plate:1
- Mate:232: .25-20 Clinch Style Pem Nut .125 Minimum Panel Thickness:2 ↔ Mounting Plate:1
- Mate:233: .25-20 Clinch Style Pem Nut .125 Minimum Panel Thickness:1 ↔ Mounting Plate:1
- Mate:234: .25-20 Clinch Style Pem Nut .125 Minimum Panel Thickness:2 ↔ Mounting Plate:1
- Mate:235: Output Shaft:1 ↔ Frame Segment:1
- Mate:236: Frame Segment:1 ↔ Mounting Plate:1
- Mate:237: Frame Segment:1 ↔ Mounting Plate:1
- Mate:238: 10-32 Clinch Style Pem Nut .091 Minimum Panel Thickness:4 ↔ Mounting Plate:1
- Mate:239: 10-32 Clinch Style Pem Nut .091 Minimum Panel Thickness:8 ↔ Mounting Plate:1
- Mate:240: Mounting Plate:1 ↔ Main Connecting Standoff:8
- Mate:241: Mounting Plate:1 ↔ Main Connecting Standoff:9
- Mate:242: Cim Plate:1 ↔ Sheild:1
- Mate:243: Cim Plate:1 ↔ Sheild:1
- Flush:3: Cim Plate:1 ↔ Sheild:1
- Mate:244: Cim Plate:1 ↔ Sheild:1
- Mate:245: Button Head Cap Screw 4-40 Thread .125 Length:7 ↔ Mounting Plate:1
- Mate:246: Cim Plate:1 ↔ Button Head Cap Screw 4-40 Thread .125 Length:4
- Mate:247: Sheild:1 ↔ Button Head Cap Screw 4-40 Thread .125 Length:4
- Mate:248: Sheild:1 ↔ Button Head Cap Screw 4-40 Thread .125 Length:7
- Mate:249: Button Head Cap Screw 4-40 Thread .125 Length:3 ↔ Mounting Plate:1
- Mate:250: Cim Plate:1 ↔ Button Head Cap Screw 4-40 Thread .125 Length:6
- Mate:251: Sheild:1 ↔ Button Head Cap Screw 4-40 Thread .125 Length:6
- Mate:252: Sheild:1 ↔ Button Head Cap Screw 4-40 Thread .125 Length:3
- Mate:253: Button Head Cap Screw 4-40 Thread .125 Length:8 ↔ Mounting Plate:1
- Mate:254: Cim Plate:1 ↔ Button Head Cap Screw 4-40 Thread .125 Length:10
- Mate:255: Sheild:1 ↔ Button Head Cap Screw 4-40 Thread .125 Length:8
- Mate:256: Sheild:1 ↔ Button Head Cap Screw 4-40 Thread .125 Length:10
- Mate:257: Button Head Cap Screw 4-40 Thread .125 Length:5 ↔ Mounting Plate:1
- Mate:258: Cim Plate:1 ↔ Button Head Cap Screw 4-40 Thread .125 Length:9
- Mate:259: Sheild:1 ↔ Button Head Cap Screw 4-40 Thread .125 Length:5
- Mate:260: Sheild:1 ↔ Button Head Cap Screw 4-40 Thread .125 Length:9
- Mate:261: Sheild:1 ↔ Sheild - Upper:1
- Flush:4: Sheild:1 ↔ Sheild - Upper:1
- Mate:262: Sheild:1 ↔ Sheild - Upper:1
